# Autodesk Inventor assembly: Assembly146-01
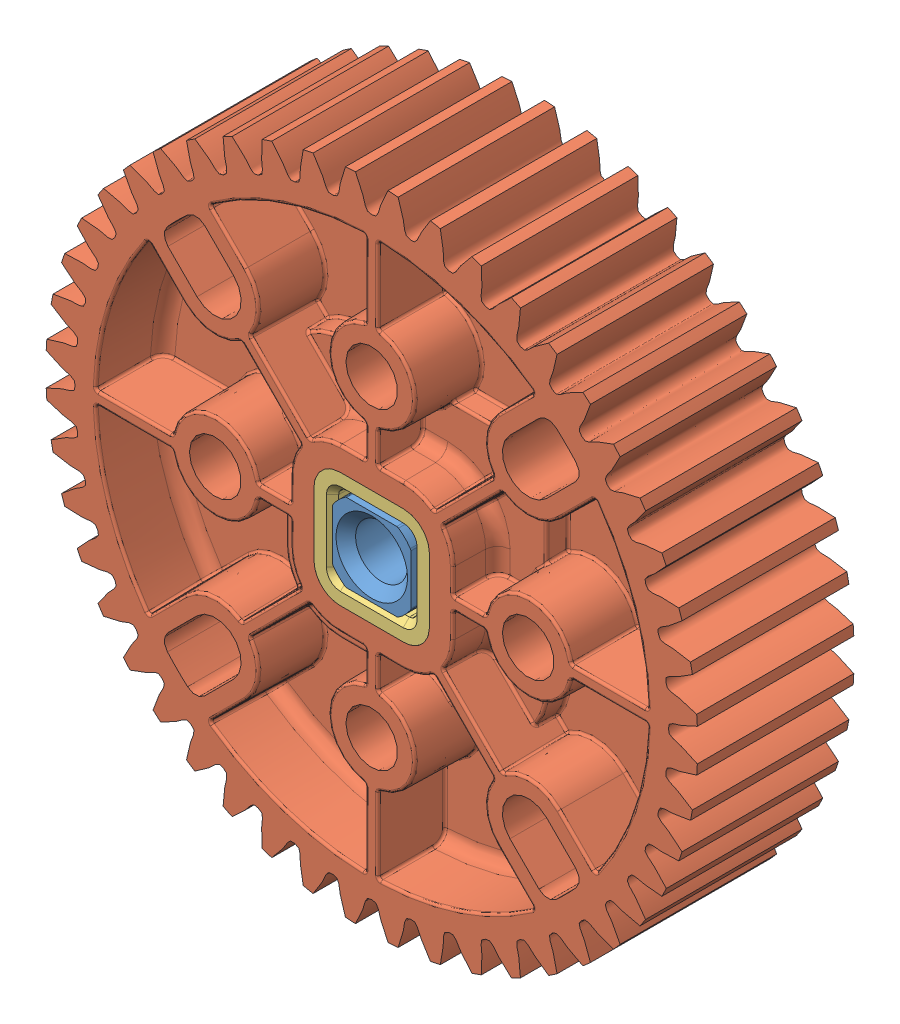
[picture p0: shaded view drawn from the shape stored in the file]
Saved by Autodesk Inventor 2026.2 (Build 302298000, 298)
## iProperties
Created: 2022-08-02
Part Number: Assembly146-01
Document SubType Name: Assembly
Designer: ylu12
Author: ylu12
## Documents named in this file (4)
- C:\Personal\Deprecated\VEX V5 Push Back\S-bot-two\CAD\VEX-CAD-Inventor-1.4.2\Motion\Gears\HS Gear\HS 48T Gear, Circle.iam
- C:\Personal\Deprecated\VEX V5 Push Back\S-bot-two\CAD\VEX-CAD-Inventor-1.4.2\Motion\HS Shaft Adapter Circle.ipt
- C:\Personal\Deprecated\VEX V5 Push Back\S-bot-two\CAD\VEX-CAD-Inventor-1.4.2\Motion\Gears\Reference Files\HS 48T Gear, No Insert.ipt
- C:\Personal\Deprecated\VEX V5 Push Back\S-bot-two\CAD\VEX-CAD-Inventor-1.4.2\Motion\Gears\HS Gear.iam
## Components (2 placed, 2 different names)
1. Circle — Mate:1, Mate:2, Flush:1
2. 48T — Flush:6, Mate:11, Mate:12
## Relationships (6: Mate 4, Flush 2)
- Mate:1: Circle
- Mate:2: Circle
- Flush:1 (6.35 mm): Circle
- Flush:6: 48T
- Mate:11: 48T
- Mate:12: 48T
